# Autodesk Inventor assembly: RobotV1
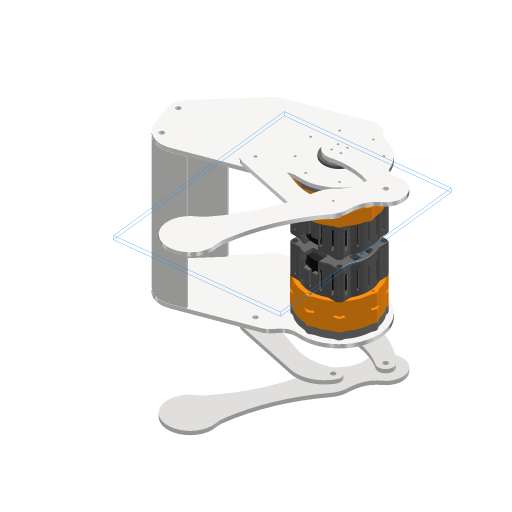
[picture p0: Inventor's stored thumbnail of the model, 512x512]
Saved by Autodesk Inventor 2024.3 (Build 283343000, 343)
## iProperties
Created: 2025-09-30
Part Number: RobotV1
Document SubType Name: Assembly
Designer: danie
Author: danie
## Documents named in this file (9)
- C:\Users\danie\OneDrive\Documentos\Inventor\Motor_drive\RobotV1.iam
- C:\Users\danie\OneDrive\Documentos\Inventor\Motor_drive\Ensamble.iam
- C:\Users\danie\OneDrive\Documentos\Inventor\Motor_drive\chasis lateral.ipt
- C:\Users\danie\OneDrive\Documentos\Inventor\Motor_drive\Link1V1.ipt
- C:\Users\danie\OneDrive\Documentos\Inventor\Motor_drive\Link2V1.ipt
- C:\Users\danie\OneDrive\Documentos\Inventor\Motor_drive\Link3V1.ipt
- C:\Users\danie\OneDrive\Documentos\Inventor\Motor_drive\Link1V1R.ipt
- C:\Users\danie\OneDrive\Documentos\Inventor\Motor_drive\frontal.ipt
- C:\Users\danie\OneDrive\Documentos\Inventor\Motor_drive\CR 30x42x7\CR 30x42x7\CR 30x42x7.ipt
## Components (12 placed, 8 different names)
1. Ensamble:2 [sub-assembly] — Mate:1, Mate:2, Flush:1, Mate:3, Mate:4, Mate:5, Mate:6, Mate:7, Mate:12, Flush:2
2. chasis lateral:1 — Mate:3, Mate:4, Mate:5, Mate:13, Mate:14, Mate:15, Mate:30, Mate:31, Mate:33
3. chasis lateral:2 — Mate:8, Mate:9, Mate:10, Mate:19, Mate:21, Mate:22
4. Ensamble:3 [sub-assembly] — Mate:6, Mate:7, Mate:8, Mate:9, Mate:10, Mate:20, Mate:23
5. Link1V1:1 — Mate:12, Mate:13, Mate:16, Mate:18, Mate:32
6. Link2V1:1 — Mate:14, Mate:15, Mate:17
7. Link3V1:1 — Mate:16, Mate:17, Mate:18, Mate:27, Mate:29
8. Link1V1R:1 — Mate:19, Mate:20, Mate:24, Mate:26, Mate:29
9. Link2V1:2 — Mate:21, Mate:22, Mate:25
10. Link3V1:2 — Mate:24, Mate:25, Mate:26, Mate:28
11. frontal:1 — Mate:30, Mate:31
12. CR 30x42x7:1 — Mate:32, Mate:33
## Relationships (34: Mate 32, Flush 2)
- Mate:1: Ensamble:2
- Mate:2: Ensamble:2
- Flush:1: Ensamble:2
- Mate:3: Ensamble:2 ↔ chasis lateral:1
- Mate:4: Ensamble:2 ↔ chasis lateral:1
- Mate:5: Ensamble:2 ↔ chasis lateral:1
- Mate:6: Ensamble:2 ↔ Ensamble:3
- Mate:7: Ensamble:2 ↔ Ensamble:3
- Mate:8: chasis lateral:2 ↔ Ensamble:3
- Mate:9: chasis lateral:2 ↔ Ensamble:3
- Mate:10: chasis lateral:2 ↔ Ensamble:3
- Mate:12: Ensamble:2 ↔ Link1V1:1
- Mate:13: chasis lateral:1 ↔ Link1V1:1
- Mate:14: chasis lateral:1 ↔ Link2V1:1
- Mate:15: chasis lateral:1 ↔ Link2V1:1
- Mate:16: Link1V1:1 ↔ Link3V1:1
- Mate:17: Link2V1:1 ↔ Link3V1:1
- Mate:18: Link1V1:1 ↔ Link3V1:1
- Mate:19: chasis lateral:2 ↔ Link1V1R:1
- Mate:20: Ensamble:3 ↔ Link1V1R:1
- Mate:21: chasis lateral:2 ↔ Link2V1:2
- Mate:22: chasis lateral:2 ↔ Link2V1:2
- Flush:2 (9.6 mm): Ensamble:2
- Mate:23: Ensamble:3
- Mate:24: Link1V1R:1 ↔ Link3V1:2
- Mate:25: Link2V1:2 ↔ Link3V1:2
- Mate:26: Link1V1R:1 ↔ Link3V1:2
- Mate:27: Link3V1:1
- Mate:28: Link3V1:2
- Mate:29: Link3V1:1 ↔ Link1V1R:1
- Mate:30: chasis lateral:1 ↔ frontal:1
- Mate:31: chasis lateral:1 ↔ frontal:1
- Mate:32: Link1V1:1 ↔ CR 30x42x7:1
- Mate:33: chasis lateral:1 ↔ CR 30x42x7:1
